# Autodesk Inventor assembly: Hub Mount
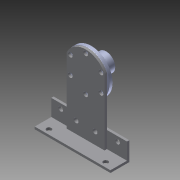
[picture p0: Inventor's stored thumbnail of the model, 180x180]
Saved by Autodesk Inventor 2014 SP1 (Build 180222100, 222)
## iProperties
Created: 2014-01-16
Part Number: Hub Mount
Document SubType Name: Assembly
Designer: JU BRIAN
Author: JU BRIAN
## Documents named in this file (4)
- K:\MHS\Technology\Holliday B\Group Projects\Robotics\CAD Team\CAD Team 2014\Chassis 2014\Hub Mount.iam
- K:\MHS\Technology\Holliday B\Group Projects\Robotics\CAD Team\CAD Team 2014\Chassis 2014\Hub Mount L Bracket.ipt
- K:\MHS\Technology\Holliday B\Group Projects\Robotics\CAD Team\CAD Team 2014\Chassis 2014\Hub Mount Plate.ipt
- K:\MHS\Technology\Holliday B\Group Projects\Robotics\CAD Team\CAD Team 2014\Chassis 2014\Imported Components\am-0077a-500 Key Hub r2\am-0077a-500 Key Hub r2.ipt
## Components (3 placed, 3 different names)
1. Hub Mount L Bracket:1 — Insert:1, Insert:2
2. Hub Mount Plate:1 — Insert:1, Insert:2, Insert:3, Insert:4
3. am-0077a-500 Key Hub r2:1 — Insert:3, Insert:4
## Relationships (4: Insert 4)
- Insert:1: Hub Mount L Bracket:1 ↔ Hub Mount Plate:1
- Insert:2: Hub Mount L Bracket:1 ↔ Hub Mount Plate:1
- Insert:3: Hub Mount Plate:1 ↔ am-0077a-500 Key Hub r2:1
- Insert:4: Hub Mount Plate:1 ↔ am-0077a-500 Key Hub r2:1
